# Autodesk Inventor assembly: pulley 48 tooth + hub_MIR
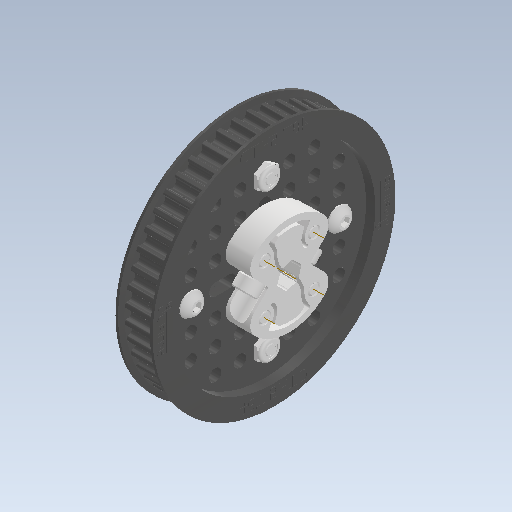
[picture p0: Inventor's stored thumbnail of the model, 512x512]
Saved by Autodesk Inventor 2020 (Build 240168000, 168)
## iProperties
Created: 2020-02-22
Part Number: pulley 48 tooth + hub_MIR
Document SubType Name: Assembly
Designer: jackm
Author: ball
## Documents named in this file (4)
- D:\FTC8863\2019 Robot\Mecanum Drive Train Metal\pulley 48 tooth + hub_MIR.iam
- D:\FTC8863\GoBilda\3415 Parts\3415-0014-0048 Assembly_MIR.ipt
- D:\FTC8863\GoBilda\1309 Parts\1309-0016-4008 assembly_MIR.ipt
- D:\FTC8863\StepLibraries\Screws\M4 x 14 BUTTON HEAD HEX DRIVE SCREW_MIR.ipt
## Components (6 placed, 3 different names)
1. 3415-0014-0048 Assembly_MIR:1 — Flush:1, Mate:2, Mate:1, Mate:9, Mate:11, Mate:15, Mate:13
2. 1309-0016-4008 assembly_MIR:1 — Flush:1, Mate:2, Mate:1, Mate:10, Mate:12, Mate:16, Mate:14
3. M4 x 14 BUTTON HEAD HEX DRIVE SCREW_MIR:1 — Mate:10, Mate:9
4. M4 x 14 BUTTON HEAD HEX DRIVE SCREW_MIR:2 — Mate:12, Mate:11
5. M4 x 14 BUTTON HEAD HEX DRIVE SCREW_MIR:3 — Mate:16, Mate:15
6. M4 x 14 BUTTON HEAD HEX DRIVE SCREW_MIR:4 — Mate:14, Mate:13
## Relationships (11: Mate 10, Flush 1)
- Flush:1: 3415-0014-0048 Assembly_MIR:1 ↔ 1309-0016-4008 assembly_MIR:1
- Mate:2: 3415-0014-0048 Assembly_MIR:1 ↔ 1309-0016-4008 assembly_MIR:1
- Mate:1: 3415-0014-0048 Assembly_MIR:1 ↔ 1309-0016-4008 assembly_MIR:1
- Mate:10: 1309-0016-4008 assembly_MIR:1 ↔ M4 x 14 BUTTON HEAD HEX DRIVE SCREW_MIR:1
- Mate:9: 3415-0014-0048 Assembly_MIR:1 ↔ M4 x 14 BUTTON HEAD HEX DRIVE SCREW_MIR:1
- Mate:12: 1309-0016-4008 assembly_MIR:1 ↔ M4 x 14 BUTTON HEAD HEX DRIVE SCREW_MIR:2
- Mate:11: 3415-0014-0048 Assembly_MIR:1 ↔ M4 x 14 BUTTON HEAD HEX DRIVE SCREW_MIR:2
- Mate:16: 1309-0016-4008 assembly_MIR:1 ↔ M4 x 14 BUTTON HEAD HEX DRIVE SCREW_MIR:3
- Mate:15: 3415-0014-0048 Assembly_MIR:1 ↔ M4 x 14 BUTTON HEAD HEX DRIVE SCREW_MIR:3
- Mate:14: 1309-0016-4008 assembly_MIR:1 ↔ M4 x 14 BUTTON HEAD HEX DRIVE SCREW_MIR:4
- Mate:13: 3415-0014-0048 Assembly_MIR:1 ↔ M4 x 14 BUTTON HEAD HEX DRIVE SCREW_MIR:4
